# Autodesk Inventor assembly: Redesign_GripperASSEM
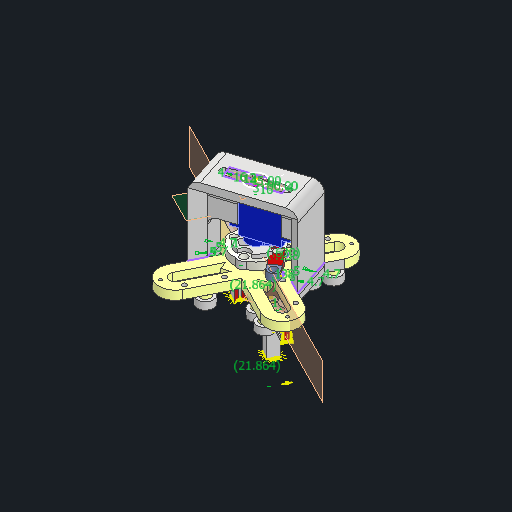
[picture p0: Inventor's stored thumbnail of the model, 512x512]
Saved by Autodesk Inventor 2025.1 (Build 291241000, 241)
## iProperties
Created: 2024-12-20
Part Number: Redesign_GripperASSEM
Document SubType Name: Assembly
Designer: m_kni
Author: m_kni
## Documents named in this file (8)
- C:\Users\jerem\Documents\GitHub\Perovskite-Automated-Synthesis-System\CAD\Gripper\Redesign_GripperASSEM.iam
- C:\Users\jerem\Documents\GitHub\Perovskite-Automated-Synthesis-System\CAD\Gripper\Redesign_Gripper_Baseplate.ipt
- C:\Users\jerem\Documents\GitHub\Perovskite-Automated-Synthesis-System\CAD\Gripper\5x5x11bearing.ipt
- C:\Users\jerem\Documents\GitHub\Perovskite-Automated-Synthesis-System\CAD\Gripper\Redesign_Gripper_Finger.ipt
- C:\Users\jerem\Documents\GitHub\Perovskite-Automated-Synthesis-System\CAD\Gripper\Redesign_Spinner.ipt
- C:\Users\jerem\Documents\GitHub\Perovskite-Automated-Synthesis-System\CAD\Non 3D Printed Parts\Motors and Servos\SG90 Servo.ipt
- C:\Users\jerem\Documents\GitHub\Perovskite-Automated-Synthesis-System\CAD\Gripper\Overhead_Bracket.ipt
- C:\Users\jerem\Documents\GitHub\Perovskite-Automated-Synthesis-System\CAD\Gripper\link assem.iam
## Components (20 placed, 7 different names)
1. Redesign_Gripper_Baseplate:1 — Insert:1, Insert:2, Insert:3, Insert:4, Insert:5, Insert:6, Insert:7, Insert:8, Insert:9, Insert:11, Insert:12, Insert:13, Flush:1, Insert:23, Angle:1
2. 5x5x11bearing:1 — Insert:7
3. 5x5x11bearing:2 — Insert:8
4. 5x5x11bearing:3 — Insert:5
5. 5x5x11bearing:4 — Insert:1
6. 5x5x11bearing:5 — Insert:2
7. 5x5x11bearing:6 — Insert:3
8. 5x5x11bearing:7 — Insert:4
9. 5x5x11bearing:8
10. 5x5x11bearing:9 — Insert:6
11. 5x5x11bearing:10 — Insert:12
12. 5x5x11bearing:11 — Insert:11
13. 5x5x11bearing:12 — Insert:9
14. Redesign_Gripper_Finger:1 — Mate:2
15. Redesign_Gripper_Finger:4
16. 5x5x11bearing:13 — Insert:13, Insert:14
17. Redesign_Spinner:1 — Insert:14, Mate:1
18. SG90 Servo:1 — Insert:22
19. Overhead_Bracket:1 — Insert:22, Insert:23, Angle:1
20. link assem:1 [sub-assembly] — Mate:1, Mate:2
## Relationships (19: Insert 15, Mate 2, Flush 1, Angle 1)
- Insert:1: Redesign_Gripper_Baseplate:1 ↔ 5x5x11bearing:4
- Insert:2: Redesign_Gripper_Baseplate:1 ↔ 5x5x11bearing:5
- Insert:3: Redesign_Gripper_Baseplate:1 ↔ 5x5x11bearing:6
- Insert:4: Redesign_Gripper_Baseplate:1 ↔ 5x5x11bearing:7
- Insert:5: Redesign_Gripper_Baseplate:1 ↔ 5x5x11bearing:3
- Insert:6: Redesign_Gripper_Baseplate:1 ↔ 5x5x11bearing:9
- Insert:7: Redesign_Gripper_Baseplate:1 ↔ 5x5x11bearing:1
- Insert:8: Redesign_Gripper_Baseplate:1 ↔ 5x5x11bearing:2
- Insert:9: Redesign_Gripper_Baseplate:1 ↔ 5x5x11bearing:12
- Insert:11: Redesign_Gripper_Baseplate:1 ↔ 5x5x11bearing:11
- Insert:12: Redesign_Gripper_Baseplate:1 ↔ 5x5x11bearing:10
- Insert:13: Redesign_Gripper_Baseplate:1 ↔ 5x5x11bearing:13
- Insert:14: 5x5x11bearing:13 ↔ Redesign_Spinner:1
- Flush:1: Redesign_Gripper_Baseplate:1
- Insert:22: SG90 Servo:1 ↔ Overhead_Bracket:1
- Insert:23: Redesign_Gripper_Baseplate:1 ↔ Overhead_Bracket:1
- Angle:1 (0 deg): Redesign_Gripper_Baseplate:1 ↔ Overhead_Bracket:1
- Mate:1: Redesign_Spinner:1 ↔ link assem:1
- Mate:2: Redesign_Gripper_Finger:1 ↔ link assem:1
